# Autodesk Inventor assembly: DriveSide
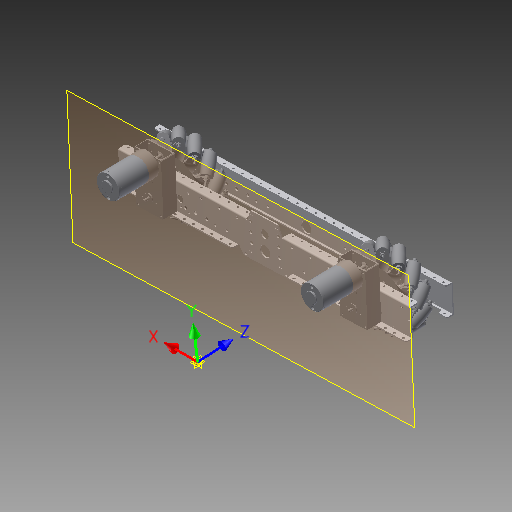
[picture p0: Inventor's stored thumbnail of the model, 512x512]
Saved by Autodesk Inventor 2018 (Build 220112000, 112)
## iProperties
Created: 2016-01-10
Part Number: DriveSide
Document SubType Name: Assembly
Designer: Applefamily
Author: Applefamily
## Documents named in this file (8)
- C:\Users\Apple\Documents\Inventor\2018 PowerUp\2016_Files_2018_Mod\Assembly\DriveSide.iam
- C:\Users\Apple\Documents\Inventor\2018 PowerUp\2016_Files_2018_Mod\Assembly\Imported Components\am-2951 AM14U2 Outside Sheet.ipt\am-2951 AM14U2 Outside Sheet.ipt.ipt
- C:\Users\Apple\Documents\Inventor\2018 PowerUp\2016_Files_2018_Mod\Assembly\GearBox and Mec.iam
- C:\Users\Apple\Documents\Inventor\2018 PowerUp\2016_Files_2018_Mod\Assembly\Imported Components\FR8ZZ Hex Bearing.ipt\FR8ZZ Hex Bearing.ipt.ipt
- C:\Users\Apple\Documents\Inventor\2018 PowerUp\2016_Files_2018_Mod\Assembly\Imported Components\am-2952 AM14U2 Inside Sheet.ipt\am-2952 AM14U2 Inside Sheet.ipt.ipt
- am-2951 AM14U2 Outside Sheet.ipt
- FR8ZZ Hex Bearing.ipt
- am-2952 AM14U2 Inside Sheet.ipt
## Components (6 placed, 4 different names)
1. am-2951 AM14U2 Outside Sheet.ipt:1 — Cylindrical:1, Cylindrical:2, Mate:1, Mate:2
2. GearBox and Mec:1 [sub-assembly] — Flush:1, Mate:3
3. FR8ZZ Hex Bearing.ipt:1 — Cylindrical:1, Mate:1
4. FR8ZZ Hex Bearing.ipt:2 — Cylindrical:2, Mate:2, Cylindrical:3
5. GearBox and Mec:2 [sub-assembly] — Cylindrical:3, Cylindrical:5, Flush:1, Mate:4
6. am-2952 AM14U2 Inside Sheet.ipt:1 — Cylindrical:5, Mate:3, Mate:4
## Relationships (9: CylindricalJoint 4, Mate 4, Flush 1)
- Cylindrical:1: am-2951 AM14U2 Outside Sheet.ipt:1 ↔ FR8ZZ Hex Bearing.ipt:1
- Cylindrical:2: am-2951 AM14U2 Outside Sheet.ipt:1 ↔ FR8ZZ Hex Bearing.ipt:2
- Mate:1: am-2951 AM14U2 Outside Sheet.ipt:1 ↔ FR8ZZ Hex Bearing.ipt:1
- Mate:2: am-2951 AM14U2 Outside Sheet.ipt:1 ↔ FR8ZZ Hex Bearing.ipt:2
- Cylindrical:3: FR8ZZ Hex Bearing.ipt:2 ↔ GearBox and Mec:2
- Cylindrical:5: GearBox and Mec:2 ↔ am-2952 AM14U2 Inside Sheet.ipt:1
- Flush:1: GearBox and Mec:1 ↔ GearBox and Mec:2
- Mate:3: GearBox and Mec:1 ↔ am-2952 AM14U2 Inside Sheet.ipt:1
- Mate:4: GearBox and Mec:2 ↔ am-2952 AM14U2 Inside Sheet.ipt:1
